# Autodesk Inventor assembly: Koruza 2
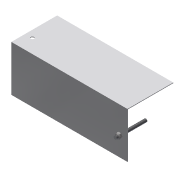
[picture p0: Inventor's stored thumbnail of the model, 180x180]
Saved by Autodesk Inventor 2015 (Build 190159000, 159)
## iProperties
Created: 2015-01-08
Part Number: Koruza 2
Document SubType Name: Assembly
Designer: Michal
Author: Michal
## Documents named in this file (4)
- C:\Users\Michal\Desktop\Michal\Prace\koruza\Koruza 2.iam
- C:\Users\Michal\Desktop\Michal\Prace\koruza\L profil.ipt
- C:\Users\Michal\Desktop\Michal\Prace\koruza\Závitová tyč M10 x 80.ipt
- C:\Users\Michal\Desktop\Michal\Prace\koruza\ANSI B18.16.3M - Property Class 5 and 10 - Metric M10 x 1.5 Typ kovu.ipt
## Components (4 placed, 3 different names)
1. L profil:1 — Proti sobě:1, Stejný směr:1, Proti sobě:3, Proti sobě:5
2. Závitová tyč M10 x 80:1 — Proti sobě:1, Stejný směr:1, Proti sobě:2, Proti sobě:4
3. ANSI B18.16.3M - Property Class 5 and 10 - Metric M10 x 1.5 Typ kovu:1 — Proti sobě:2, Proti sobě:3
4. ANSI B18.16.3M - Property Class 5 and 10 - Metric M10 x 1.5 Typ kovu:2 — Proti sobě:4, Proti sobě:5
## Relationships (6: Mate 5, Flush 1)
- Proti sobě:1 [Mate]: L profil:1 ↔ Závitová tyč M10 x 80:1
- Stejný směr:1 [Flush] (15 mm): L profil:1 ↔ Závitová tyč M10 x 80:1
- Proti sobě:2 [Mate]: Závitová tyč M10 x 80:1 ↔ ANSI B18.16.3M - Property Class 5 and 10 - Metric M10 x 1.5 Typ kovu:1
- Proti sobě:3 [Mate]: L profil:1 ↔ ANSI B18.16.3M - Property Class 5 and 10 - Metric M10 x 1.5 Typ kovu:1
- Proti sobě:4 [Mate]: Závitová tyč M10 x 80:1 ↔ ANSI B18.16.3M - Property Class 5 and 10 - Metric M10 x 1.5 Typ kovu:2
- Proti sobě:5 [Mate]: L profil:1 ↔ ANSI B18.16.3M - Property Class 5 and 10 - Metric M10 x 1.5 Typ kovu:2
